# Autodesk Inventor assembly: manipulator
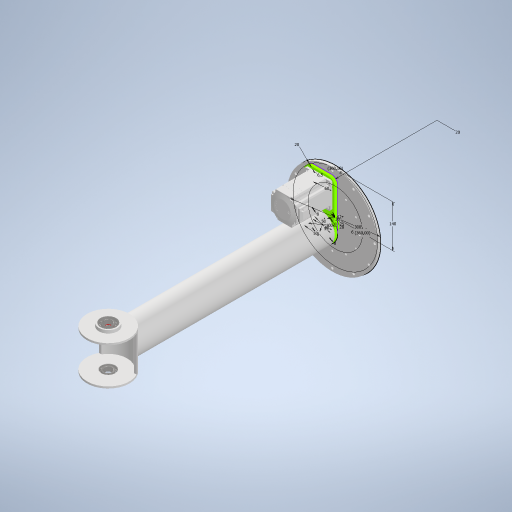
[picture p0: Inventor's stored thumbnail of the model, 512x512]
Saved by Autodesk Inventor 2023 (Build 270158000, 158)
## iProperties
Created: 2023-03-28
Part Number: manipulator
Document SubType Name: Assembly
Designer: krzys
Author: krzys
## Documents named in this file (12)
- C:\Users\Wiktor\Documents\Manipulator\Manipulator.iam
- C:\Users\Wiktor\Documents\Manipulator\podstawa.ipt
- C:\Users\Wiktor\Documents\Manipulator\manipulator\Design Accelerator\Łożysko1.iam
- C:\Users\Wiktor\Documents\Manipulator\tuleja_dystansowa.ipt
- C:\Users\Wiktor\Documents\Manipulator\podstwa_obrotowa.ipt
- C:\Users\Wiktor\Documents\Manipulator\CS-M23480_3D.ipt
- C:\Users\Wiktor\Documents\Manipulator\czlon1.ipt
- C:\Users\Wiktor\Documents\Manipulator\czlon_1.ipt
- C:\Users\Wiktor\Documents\Manipulator\manipulator\Design Accelerator\Łożysko3.iam
- C:\Users\Wiktor\Documents\Manipulator\Manipulator\Design Accelerator\Łożysko2.iam
- C:\Users\Wiktor\Documents\Manipulator\Manipulator\Design Accelerator\Łożysko4.iam
- C:\Users\Wiktor\Documents\Manipulator\Gotowa przekładnia.iam
## Components (13 placed, 8 different names)
1. podstawa:1
2. Łożysko:1 [sub-assembly]
3. Łożysko:2 [sub-assembly]
4. tuleja_dystansowa:1
5. podstwa_obrotowa:1
6. CS-M23480_3D:1
7. czlon1:1
8. czlon_1:1 — Zestawiające:1, Zestawiające:2, Zestawiające:3, Zestawiające:4, Zestawiające:5
9. Łożysko:3 [sub-assembly]
10. Łożysko:4 [sub-assembly]
11. Łożysko:5 [sub-assembly] — Zestawiające:1, Zestawiające:2, Zestawiające:6
12. Łożysko:6 [sub-assembly] — Zestawiające:3, Zestawiające:4
13. Gotowa przekładnia:1 [sub-assembly] — Zestawiające:5, Zestawiające:6
## Relationships (6: Mate 6)
- Zestawiające:1 [Mate]: czlon_1:1 ↔ Łożysko:5
- Zestawiające:2 [Mate]: czlon_1:1 ↔ Łożysko:5
- Zestawiające:3 [Mate]: czlon_1:1 ↔ Łożysko:6
- Zestawiające:4 [Mate]: czlon_1:1 ↔ Łożysko:6
- Zestawiające:5 [Mate]: czlon_1:1 ↔ Gotowa przekładnia:1
- Zestawiające:6 [Mate]: Łożysko:5 ↔ Gotowa przekładnia:1
